# Autodesk Inventor assembly: gate_nor
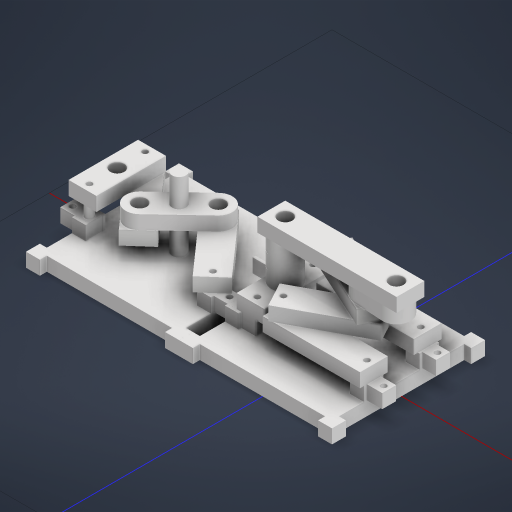
[picture p0: Inventor's stored thumbnail of the model, 512x512]
Saved by Autodesk Inventor 2024.3 (Build 283343000, 343)
## iProperties
Created: 2024-09-29
Part Number: gate_nor
Document SubType Name: Assembly
Designer: sam
Author: sam
## Documents named in this file (3)
- N:\Cad\computer\gates\gate_nor.iam
- N:\Cad\computer\gates\gate_not.iam
- N:\Cad\computer\gates\gate_or.iam
## Components (2 placed, 2 different names)
1. gate_not:1 [sub-assembly] — Mate:1, Flush:1, Flush:2, Mate:2
2. gate_or:1 [sub-assembly] — Mate:1, Flush:1, Flush:2, Mate:2
## Relationships (4: Mate 2, Flush 2)
- Mate:1: gate_not:1 ↔ gate_or:1
- Flush:1: gate_not:1 ↔ gate_or:1
- Flush:2: gate_not:1 ↔ gate_or:1
- Mate:2: gate_not:1 ↔ gate_or:1
